# Autodesk Inventor assembly: s-assy-link0
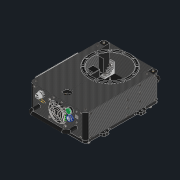
[picture p0: Inventor's stored thumbnail of the model, 180x180]
Saved by Autodesk Inventor 2022 (Build 260153000, 153)
## iProperties
Created: 2021-07-12
Part Number: s-assy-link0
Document SubType Name: Assembly
Designer: yuta0
Mass: 4333.24 g
Surface Area: 5973.62 cm^2
Volume: 1138.09 cm^3
Density: 3.80748 g/cm^3
Author: yuta0
## Documents named in this file (27)
- C:\Users\yuta0\Documents\GitHub\catchrobo_hardware\assy-robot\s-assy-link0.iam
- C:\Users\yuta0\Documents\GitHub\catchrobo_hardware\assy-robot\alminium_base1.ipt
- C:\Users\yuta0\Documents\GitHub\catchrobo_hardware\assy-robot\carbon_plate6.ipt
- C:\Users\yuta0\Documents\GitHub\catchrobo_hardware\assy-robot\carbon_plate7.ipt
- C:\Users\yuta0\Documents\GitHub\catchrobo_hardware\assy-robot\NBLTS5_b.ipt
- C:\Users\yuta0\Documents\GitHub\catchrobo_hardware\assy-robot\UWANK10-120-27.ipt
- C:\Users\yuta0\Documents\GitHub\catchrobo_hardware\assy-robot\s-assyypanel.iam
- C:\Users\yuta0\Documents\GitHub\catchrobo_hardware\assy-robot\CB5-12.ipt
- C:\Users\yuta0\Documents\GitHub\catchrobo_hardware\assy-robot\s-assy-pillar1.iam
- C:\Users\yuta0\Documents\GitHub\catchrobo_hardware\assy-robot\s-assy-pillar2.iam
- C:\Users\yuta0\Documents\GitHub\catchrobo_hardware\assy-robot\s-assy-pillar3.iam
- C:\Users\yuta0\Documents\GitHub\catchrobo_hardware\assy-robot\CB3-5.ipt
- C:\Users\yuta0\Documents\GitHub\catchrobo_hardware\assy-robot\steel_plate4.ipt
- C:\Users\yuta0\Documents\GitHub\catchrobo_hardware\assy-robot\Fullymax_6s.ipt
- C:\Users\yuta0\Documents\GitHub\catchrobo_hardware\assy-robot\ODrive3.4.ipt
- C:\Users\yuta0\Documents\GitHub\catchrobo_hardware\assy-robot\power_supply_unit.ipt
- C:\Users\yuta0\Documents\GitHub\catchrobo_hardware\assy-robot\U2H-Z7SBK.ipt
- C:\Users\yuta0\Documents\GitHub\catchrobo_hardware\assy-robot\s-assy-unit-j1.iam
- C:\Users\yuta0\Documents\GitHub\catchrobo_hardware\assy-robot\50wr5j cement resistor.ipt
- C:\Users\yuta0\Documents\GitHub\catchrobo_hardware\assy-robot\LBNR3.ipt
- C:\Users\yuta0\Documents\GitHub\catchrobo_hardware\assy-robot\CB4-10.ipt
- C:\Users\yuta0\Documents\GitHub\catchrobo_hardware\assy-robot\carbon_plate12.ipt
- C:\Users\yuta0\Documents\GitHub\catchrobo_hardware\assy-robot\hexagonal_spacer_M3_5mm.ipt
- C:\Users\yuta0\Documents\GitHub\catchrobo_hardware\assy-robot\hexagonal_spacer_M3_30mm.ipt
- C:\Users\yuta0\Documents\GitHub\catchrobo_hardware\assy-robot\s-assy-cover-right.iam
- C:\Users\yuta0\Documents\GitHub\catchrobo_hardware\assy-robot\s-assy-cover-left.iam
- C:\Users\yuta0\Documents\GitHub\catchrobo_hardware\assy-robot\base46.ipt
## Components (100 placed, 26 different names)
1. alminium_base1:2 — メイト:123, メイト:124, メイト:125, メイト:126, メイト:127, メイト:128, メイト:129, 角度:1, 角度:2, メイト:153, メイト:155, メイト:157, メイト:162, メイト:177, メイト:178, メイト:179, メイト:180, メイト:189, メイト:194, メイト:195, メイト:196, メイト:197, メイト:198, メイト:199, メイト:200, メイト:201, メイト:202, メイト:203, メイト:221, メイト:222, メイト:224, メイト:225, メイト:228, メイト:229, メイト:243, メイト:244, メイト:245, メイト:246, メイト:248, メイト:249
2. s-assy-unit-j1:1 [sub-assembly] — メイト:201, メイト:202, メイト:203, メイト:204, メイト:205, メイト:250, メイト:251, メイト:252
3. s-assy-pillar1:1 [sub-assembly] — メイト:153, メイト:159, メイト:178, メイト:240, メイト:241
4. s-assy-pillar1:2 [sub-assembly] — メイト:155, メイト:164, メイト:179, メイト:181, メイト:236
5. s-assy-pillar2:1 [sub-assembly] — メイト:157, メイト:160, メイト:161, メイト:177, メイト:183, フラッシュ:5, メイト:239, メイト:242
6. s-assy-pillar3:1 [sub-assembly] — メイト:162, メイト:165, メイト:166, メイト:180, メイト:185, メイト:237, メイト:238
7. s-assyypanel:1 [sub-assembly] — メイト:134, メイト:135, メイト:136, メイト:182
8. s-assy-cover-right:1 [sub-assembly] — メイト:236, メイト:237, メイト:238
9. s-assy-cover-left:1 [sub-assembly] — メイト:239, メイト:240, メイト:241
10. carbon_plate12:1 — メイト:159, メイト:160, メイト:161, メイト:184, メイト:193
11. carbon_plate6:2 — メイト:164, メイト:165, メイト:166, メイト:186, メイト:206, メイト:207, メイト:208, メイト:209, メイト:210, メイト:211, メイト:212, メイト:213, メイト:214, メイト:215, メイト:216
12. carbon_plate7:1 — メイト:130, メイト:131, メイト:132, メイト:133, メイト:176
13. steel_plate4:1 — メイト:189, メイト:190, メイト:191, メイト:192, フラッシュ:4, メイト:247
14. NBLTS5_b:1 — メイト:97, フラッシュ:3, メイト:124, メイト:125, メイト:131, メイト:132, メイト:139, メイト:140, メイト:143, メイト:144
15. UWANK10-120-27:1 — メイト:97, メイト:99, メイト:133
16. Fullymax_6s:1 — メイト:192, メイト:193, フラッシュ:4
17. power_supply_unit:1 — メイト:196, メイト:197, メイト:200, メイト:226, メイト:227
18. U2H-Z7SBK:1 — メイト:199, フラッシュ:5, メイト:223
19. 50wr5j cement resistor:1 — メイト:206, メイト:207, メイト:208
20. 50wr5j cement resistor:2 — メイト:209, メイト:210
21. 50wr5j cement resistor:3 — メイト:211, メイト:212, メイト:217, メイト:219
22. NBLTS5_b:2 — メイト:99, フラッシュ:3, メイト:123, メイト:130, メイト:137, メイト:138, メイト:141, メイト:142, メイト:223
23. NBLTS5_b:3 — メイト:126, メイト:127, 角度:1, メイト:134, メイト:149, メイト:150, メイト:151, メイト:152
24. NBLTS5_b:4 — メイト:128, メイト:129, 角度:2, メイト:135, メイト:136, メイト:145, メイト:146, メイト:147, メイト:148
25. CB5-12:1 — メイト:137, メイト:138
26. CB5-12:2 — メイト:139, メイト:140
27. CB5-12:3 — メイト:141, メイト:142
28. CB5-12:4 — メイト:143, メイト:144
29. CB5-12:5 — メイト:145, メイト:146
30. CB5-12:6 — メイト:147, メイト:148
31. CB5-12:7 — メイト:149, メイト:150
32. CB5-12:8 — メイト:151, メイト:152
33. ODrive3.4:1 — メイト:194, メイト:195, メイト:198, メイト:253, メイト:254
34. base46:1 — メイト:250, メイト:251, メイト:252
35. CB3-5:5 — メイト:176
36. CB3-5:6 — メイト:181, メイト:182
37. CB3-5:7
38. CB3-5:8
39. CB3-5:9 — メイト:242
40. CB3-5:10
41. CB3-5:11
42. CB3-5:12
43. CB3-5:13 — メイト:183, メイト:184
44. CB3-5:14 — メイト:185, メイト:186
45. CB3-5:15
46. CB3-5:16
47. CB3-5:17
48. CB3-5:18
49. CB3-5:19
50. CB3-5:20
51. CB3-5:21 — メイト:190, メイト:191, メイト:245
52. CB3-5:22 — メイト:246, メイト:247
53. CB3-5:23 — メイト:204, メイト:205
54. CB3-5:24
55. CB3-5:26 — メイト:215, メイト:216, メイト:220
56. CB3-5:25 — メイト:213, メイト:214, メイト:218
57. LBNR3:1 — メイト:217, メイト:218
58. LBNR3:2 — メイト:219, メイト:220
59. CB3-5:27
60. CB3-5:28
61. LBNR3:3
62. LBNR3:5
63. CB3-5:29
64. CB3-5:30
65. LBNR3:4
66. LBNR3:6
67. CB4-10:1 — メイト:221, メイト:222
68. CB4-10:2
69. CB4-10:3
70. CB4-10:4
71. CB4-10:5
72. CB4-10:6
73. CB4-10:7
74. CB4-10:8
75. CB4-10:9
76. CB4-10:10
77. CB4-10:11
78. CB4-10:12
79. hexagonal_spacer_M3_5mm:1 — メイト:224, メイト:225, 角度:6
80. CB3-5:31 — メイト:226, メイト:227
81. hexagonal_spacer_M3_5mm:2
82. CB3-5:32
83. hexagonal_spacer_M3_5mm:4
84. CB3-5:34
85. CB5-12:9 — メイト:243, メイト:244
86. CB5-12:10
87. CB5-12:11
88. CB5-12:12
89. CB3-5:39 — メイト:248, メイト:249
90. CB3-5:40
91. CB3-5:41
92. CB3-5:42
93. CB3-5:35 — メイト:253, メイト:254
94. hexagonal_spacer_M3_30mm:1 — メイト:228, メイト:229, 角度:6
95. CB3-5:43
96. hexagonal_spacer_M3_30mm:2
97. CB3-5:44
98. hexagonal_spacer_M3_30mm:3
99. CB3-5:45
100. hexagonal_spacer_M3_30mm:4
## Component patterns: (4 elements, first: CB3-5:5 + CB3-5:6), (4 elements, first: CB3-5:13 + CB3-5:14), (2 elements, first: CB3-5:21), (2 elements, first: CB3-5:23), (3 elements, first: CB3-5:26 + CB3-5:25 + LBNR3:1 + LBNR3:2), (12 elements, first: CB4-10:1), (4 elements, first: hexagonal_spacer_M3_5mm:1 + CB3-5:31), (4 elements, first: CB5-12:9), (4 elements, first: CB3-5:39), (4 elements, first: CB3-5:35 + hexagonal_spacer_M3_30mm:1)
## Relationships (119: Mate 113, Flush 3, Angle 3)
- メイト:97 [Mate]: NBLTS5_b:1 ↔ UWANK10-120-27:1
- メイト:99 [Mate]: UWANK10-120-27:1 ↔ NBLTS5_b:2
- フラッシュ:3 [Flush]: NBLTS5_b:1 ↔ NBLTS5_b:2
- メイト:123 [Mate]: alminium_base1:2 ↔ NBLTS5_b:2
- メイト:124 [Mate]: alminium_base1:2 ↔ NBLTS5_b:1
- メイト:125 [Mate]: alminium_base1:2 ↔ NBLTS5_b:1
- メイト:126 [Mate]: alminium_base1:2 ↔ NBLTS5_b:3
- メイト:127 [Mate]: alminium_base1:2 ↔ NBLTS5_b:3
- メイト:128 [Mate]: alminium_base1:2 ↔ NBLTS5_b:4
- メイト:129 [Mate]: alminium_base1:2 ↔ NBLTS5_b:4
- メイト:130 [Mate]: carbon_plate7:1 ↔ NBLTS5_b:2
- メイト:131 [Mate]: carbon_plate7:1 ↔ NBLTS5_b:1
- メイト:132 [Mate]: carbon_plate7:1 ↔ NBLTS5_b:1
- メイト:133 [Mate]: carbon_plate7:1 ↔ UWANK10-120-27:1
- 角度:1 [Angle] (0 deg): alminium_base1:2 ↔ NBLTS5_b:3
- 角度:2 [Angle] (0 deg): alminium_base1:2 ↔ NBLTS5_b:4
- メイト:134 [Mate]: s-assyypanel:1 ↔ NBLTS5_b:3
- メイト:135 [Mate]: s-assyypanel:1 ↔ NBLTS5_b:4
- メイト:136 [Mate]: s-assyypanel:1 ↔ NBLTS5_b:4
- メイト:137 [Mate]: NBLTS5_b:2 ↔ CB5-12:1
- メイト:138 [Mate]: NBLTS5_b:2 ↔ CB5-12:1
- メイト:139 [Mate]: NBLTS5_b:1 ↔ CB5-12:2
- メイト:140 [Mate]: NBLTS5_b:1 ↔ CB5-12:2
- メイト:141 [Mate]: NBLTS5_b:2 ↔ CB5-12:3
- メイト:142 [Mate]: NBLTS5_b:2 ↔ CB5-12:3
- メイト:143 [Mate]: NBLTS5_b:1 ↔ CB5-12:4
- メイト:144 [Mate]: NBLTS5_b:1 ↔ CB5-12:4
- メイト:145 [Mate]: NBLTS5_b:4 ↔ CB5-12:5
- メイト:146 [Mate]: NBLTS5_b:4 ↔ CB5-12:5
- メイト:147 [Mate]: NBLTS5_b:4 ↔ CB5-12:6
- メイト:148 [Mate]: NBLTS5_b:4 ↔ CB5-12:6
- メイト:149 [Mate]: NBLTS5_b:3 ↔ CB5-12:7
- メイト:150 [Mate]: NBLTS5_b:3 ↔ CB5-12:7
- メイト:151 [Mate]: NBLTS5_b:3 ↔ CB5-12:8
- メイト:152 [Mate]: NBLTS5_b:3 ↔ CB5-12:8
- メイト:153 [Mate]: alminium_base1:2 ↔ s-assy-pillar1:1
- メイト:155 [Mate]: alminium_base1:2 ↔ s-assy-pillar1:2
- メイト:157 [Mate]: alminium_base1:2 ↔ s-assy-pillar2:1
- メイト:159 [Mate]: s-assy-pillar1:1 ↔ carbon_plate12:1
- メイト:160 [Mate]: s-assy-pillar2:1 ↔ carbon_plate12:1
- メイト:161 [Mate]: s-assy-pillar2:1 ↔ carbon_plate12:1
- メイト:162 [Mate]: alminium_base1:2 ↔ s-assy-pillar3:1
- メイト:164 [Mate]: s-assy-pillar1:2 ↔ carbon_plate6:2
- メイト:165 [Mate]: s-assy-pillar3:1 ↔ carbon_plate6:2
- メイト:166 [Mate]: s-assy-pillar3:1 ↔ carbon_plate6:2
- メイト:176 [Mate]: carbon_plate7:1 ↔ CB3-5:5
- メイト:177 [Mate]: alminium_base1:2 ↔ s-assy-pillar2:1
- メイト:178 [Mate]: alminium_base1:2 ↔ s-assy-pillar1:1
- メイト:179 [Mate]: alminium_base1:2 ↔ s-assy-pillar1:2
- メイト:180 [Mate]: alminium_base1:2 ↔ s-assy-pillar3:1
- メイト:181 [Mate]: s-assy-pillar1:2 ↔ CB3-5:6
- メイト:182 [Mate]: s-assyypanel:1 ↔ CB3-5:6
- メイト:183 [Mate]: s-assy-pillar2:1 ↔ CB3-5:13
- メイト:184 [Mate]: carbon_plate12:1 ↔ CB3-5:13
- メイト:185 [Mate]: s-assy-pillar3:1 ↔ CB3-5:14
- メイト:186 [Mate]: carbon_plate6:2 ↔ CB3-5:14
- メイト:189 [Mate]: alminium_base1:2 ↔ steel_plate4:1
- メイト:190 [Mate]: steel_plate4:1 ↔ CB3-5:21
- メイト:191 [Mate]: steel_plate4:1 ↔ CB3-5:21
- メイト:192 [Mate]: steel_plate4:1 ↔ Fullymax_6s:1
- メイト:193 [Mate]: carbon_plate12:1 ↔ Fullymax_6s:1
- フラッシュ:4 [Flush] (25 mm): steel_plate4:1 ↔ Fullymax_6s:1
- メイト:194 [Mate]: alminium_base1:2 ↔ ODrive3.4:1
- メイト:195 [Mate]: alminium_base1:2 ↔ ODrive3.4:1
- メイト:196 [Mate]: alminium_base1:2 ↔ power_supply_unit:1
- メイト:197 [Mate]: alminium_base1:2 ↔ power_supply_unit:1
- メイト:198 [Mate] (30 mm): alminium_base1:2 ↔ ODrive3.4:1
- メイト:199 [Mate]: alminium_base1:2 ↔ U2H-Z7SBK:1
- フラッシュ:5 [Flush]: s-assy-pillar2:1 ↔ U2H-Z7SBK:1
- メイト:200 [Mate] (5 mm): alminium_base1:2 ↔ power_supply_unit:1
- メイト:201 [Mate]: alminium_base1:2 ↔ s-assy-unit-j1:1
- メイト:202 [Mate]: alminium_base1:2 ↔ s-assy-unit-j1:1
- メイト:203 [Mate]: alminium_base1:2 ↔ s-assy-unit-j1:1
- メイト:204 [Mate]: s-assy-unit-j1:1 ↔ CB3-5:23
- メイト:205 [Mate]: s-assy-unit-j1:1 ↔ CB3-5:23
- メイト:206 [Mate]: carbon_plate6:2 ↔ 50wr5j cement resistor:1
- メイト:207 [Mate]: carbon_plate6:2 ↔ 50wr5j cement resistor:1
- メイト:208 [Mate]: carbon_plate6:2 ↔ 50wr5j cement resistor:1
- メイト:209 [Mate]: carbon_plate6:2 ↔ 50wr5j cement resistor:2
- メイト:210 [Mate]: carbon_plate6:2 ↔ 50wr5j cement resistor:2
- メイト:211 [Mate]: carbon_plate6:2 ↔ 50wr5j cement resistor:3
- メイト:212 [Mate]: carbon_plate6:2 ↔ 50wr5j cement resistor:3
- メイト:213 [Mate]: carbon_plate6:2 ↔ CB3-5:25
- メイト:214 [Mate]: carbon_plate6:2 ↔ CB3-5:25
- メイト:215 [Mate]: carbon_plate6:2 ↔ CB3-5:26
- メイト:216 [Mate]: carbon_plate6:2 ↔ CB3-5:26
- メイト:217 [Mate]: 50wr5j cement resistor:3 ↔ LBNR3:1
- メイト:218 [Mate]: CB3-5:25 ↔ LBNR3:1
- メイト:219 [Mate]: 50wr5j cement resistor:3 ↔ LBNR3:2
- メイト:220 [Mate]: CB3-5:26 ↔ LBNR3:2
- メイト:221 [Mate]: alminium_base1:2 ↔ CB4-10:1
- メイト:222 [Mate]: alminium_base1:2 ↔ CB4-10:1
- メイト:223 [Mate]: U2H-Z7SBK:1 ↔ NBLTS5_b:2
- メイト:224 [Mate]: alminium_base1:2 ↔ hexagonal_spacer_M3_5mm:1
- メイト:225 [Mate]: alminium_base1:2 ↔ hexagonal_spacer_M3_5mm:1
- メイト:226 [Mate]: power_supply_unit:1 ↔ CB3-5:31
- メイト:227 [Mate]: power_supply_unit:1 ↔ CB3-5:31
- メイト:228 [Mate]: alminium_base1:2 ↔ hexagonal_spacer_M3_30mm:1
- メイト:229 [Mate]: alminium_base1:2 ↔ hexagonal_spacer_M3_30mm:1
- 角度:6 [Angle] (0 deg): hexagonal_spacer_M3_5mm:1 ↔ hexagonal_spacer_M3_30mm:1
- メイト:236 [Mate]: s-assy-pillar1:2 ↔ s-assy-cover-right:1
- メイト:237 [Mate]: s-assy-pillar3:1 ↔ s-assy-cover-right:1
- メイト:238 [Mate]: s-assy-pillar3:1 ↔ s-assy-cover-right:1
- メイト:239 [Mate]: s-assy-pillar2:1 ↔ s-assy-cover-left:1
- メイト:240 [Mate]: s-assy-pillar1:1 ↔ s-assy-cover-left:1
- メイト:241 [Mate]: s-assy-pillar1:1 ↔ s-assy-cover-left:1
- メイト:242 [Mate]: s-assy-pillar2:1 ↔ CB3-5:9
- メイト:243 [Mate]: alminium_base1:2 ↔ CB5-12:9
- メイト:244 [Mate] (6 mm): alminium_base1:2 ↔ CB5-12:9
- メイト:245 [Mate]: alminium_base1:2 ↔ CB3-5:21
- メイト:246 [Mate]: alminium_base1:2 ↔ CB3-5:22
- メイト:247 [Mate]: steel_plate4:1 ↔ CB3-5:22
- メイト:248 [Mate]: alminium_base1:2 ↔ CB3-5:39
- メイト:249 [Mate]: alminium_base1:2 ↔ CB3-5:39
- メイト:250 [Mate]: s-assy-unit-j1:1 ↔ base46:1
- メイト:251 [Mate]: s-assy-unit-j1:1 ↔ base46:1
- メイト:252 [Mate]: s-assy-unit-j1:1 ↔ base46:1
- メイト:253 [Mate]: ODrive3.4:1 ↔ CB3-5:35
- メイト:254 [Mate]: ODrive3.4:1 ↔ CB3-5:35
